# Autodesk Inventor assembly: Arm 2.0 Assembly
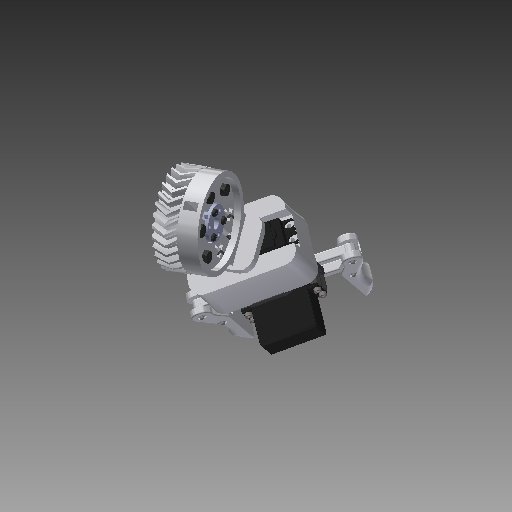
[picture p0: Inventor's stored thumbnail of the model, 512x512]
Saved by Autodesk Inventor 2017 (Build 210142000, 142)
## iProperties
Created: 2017-09-28
Part Number: Arm 2.0 Assembly
Document SubType Name: Assembly
Designer: Zach
Author: Zach
## Documents named in this file (13)
- C:\Users\Dell\Documents\GitHub\tr1\src\Body\Arm Assembly\End Effector Assembly\End Effector Assembly.iam
- C:\Users\Dell\Documents\GitHub\tr1\src\Body\Arm Assembly\End Effector Assembly\Gripper Assembly\Gripper B Assembly.iam
- C:\Users\Dell\Documents\GitHub\tr1\lib\8mm Hub.ipt
- C:\Users\Dell\Documents\GitHub\tr1\lib\Content Center Files\R2017\en-US\ISO 7045  H\ISO 7045 - M3 x 8 - 4.8 - H - ISO.ipt
- C:\Users\Dell\Documents\GitHub\tr1\src\Body\Arm Assembly\End Effector Assembly\AA046.ipt
- C:\Users\Dell\Documents\GitHub\tr1\lib\MG995.ipt
- C:\Users\Dell\Documents\GitHub\tr1\lib\Servo Mounting Hub.ipt
- C:\Users\Dell\Documents\GitHub\tr1\src\Body\Arm Assembly\End Effector Assembly\AA047.ipt
- C:\Users\Dell\Documents\GitHub\tr1\src\Body\Arm Assembly\End Effector Assembly\AA048.ipt
- C:\Users\Dell\Documents\GitHub\tr1\lib\Content Center Files\R2017\en-US\ISO 4018\ISO 4018 - M5 x 10.ipt
- C:\Users\Dell\Documents\GitHub\tr1\lib\Content Center Files\R2017\en-US\ISO 4018\ISO 4018 - M5 x 25.ipt
- C:\Users\Dell\Documents\GitHub\tr1\lib\Content Center Files\R2017\en-US\ISO 7045  H\ISO 7045 - M3 x 12 - 4.8 - H - ISO.ipt
- C:\Users\Dell\Documents\GitHub\tr1\src\Body\Arm Assembly\End Effector Assembly\AASG09b.ipt
## Components (22 placed, 12 different names)
1. AA046:1 — Mate:727, Mate:728, Mate:735, Mate:736, Mate:737, Mate:752, Mate:756, Mate:760, Mate:1298, Mate:1299, Mate:1300, Mate:1301, Mate:1302, Mate:1303, Mate:1304, Mate:1305
2. AA047:1 — Mate:735, Mate:736, Mate:737, Mate:738, Mate:739, Mate:740, Mate:753, Mate:754, Mate:755, Mate:800, Mate:801
3. AA048:1 — Mate:744, Mate:745, Mate:746, Mate:747, Mate:748, Mate:749
4. Gripper B Assembly:1 [sub-assembly] — Mate:747, Mate:748, Mate:749
5. 8mm Hub:9 — Mate:727, Mate:728, Mate:756, Mate:764, Mate:765, Mate:766, Mate:767, Mate:768, Mate:769
6. Servo Mounting Hub:1 — Mate:733, Mate:734, Mate:738, Mate:739, Mate:740, Mate:792, Mate:793, Mate:794, Mate:795, Mate:796, Mate:797, Mate:798, Mate:799
7. MG995:1 — Mate:733, Mate:734, Mate:744, Mate:745, Mate:746
8. ISO 7045 H M3 x 8 - 4.8 - H:7 — Mate:795, Mate:799
9. ISO 7045 H M3 x 8 - 4.8 - H:8 — Mate:794, Mate:798
10. ISO 7045 H M3 x 8 - 4.8 - H:9 — Mate:792, Mate:796
11. ISO 7045 H M3 x 8 - 4.8 - H:10 — Mate:793, Mate:797
12. ISO 7045 H M3 x 8 - 4.8 - H:11 — Mate:800, Mate:801
13. ISO 7045 H M3 x 12 - 4.8 - H:1 — Mate:765, Mate:767
14. ISO 7045 H M3 x 12 - 4.8 - H:3 — Mate:764, Mate:769
15. ISO 7045 H M3 x 12 - 4.8 - H:2 — Mate:766, Mate:768
16. ISO 4018 M5 x 10:1 — Mate:754, Mate:755
17. ISO 4018 M5 x 10:2 — Mate:752, Mate:753
18. ISO 4018 M5 x 25:1 — Mate:1299, Mate:1300
19. ISO 4018 M5 x 25:2 — Mate:1298, Mate:1301, Mate:1306
20. ISO 4018 M5 x 25:3 — Mate:760, Mate:1302
21. ISO 4018 M5 x 25:7 — Mate:1303, Mate:1304, Mate:1307
22. Spur Gear1:1 — Mate:1305, Mate:1306, Mate:1307
## Relationships (48: Mate 48)
- Mate:727: AA046:1 ↔ 8mm Hub:9
- Mate:728: AA046:1 ↔ 8mm Hub:9
- Mate:733: Servo Mounting Hub:1 ↔ MG995:1
- Mate:734: Servo Mounting Hub:1 ↔ MG995:1
- Mate:735: AA046:1 ↔ AA047:1
- Mate:736: AA046:1 ↔ AA047:1
- Mate:737: AA046:1 ↔ AA047:1
- Mate:738: AA047:1 ↔ Servo Mounting Hub:1
- Mate:739: AA047:1 ↔ Servo Mounting Hub:1
- Mate:740: AA047:1 ↔ Servo Mounting Hub:1
- Mate:744: AA048:1 ↔ MG995:1
- Mate:745 (0.5 mm): AA048:1 ↔ MG995:1
- Mate:746 (0.5 mm): AA048:1 ↔ MG995:1
- Mate:747: AA048:1 ↔ Gripper B Assembly:1
- Mate:748: AA048:1 ↔ Gripper B Assembly:1
- Mate:749: AA048:1 ↔ Gripper B Assembly:1
- Mate:752: AA046:1 ↔ ISO 4018 M5 x 10:2
- Mate:753: AA047:1 ↔ ISO 4018 M5 x 10:2
- Mate:754: AA047:1 ↔ ISO 4018 M5 x 10:1
- Mate:755: AA047:1 ↔ ISO 4018 M5 x 10:1
- Mate:756: AA046:1 ↔ 8mm Hub:9
- Mate:760: AA046:1 ↔ ISO 4018 M5 x 25:3
- Mate:764: 8mm Hub:9 ↔ ISO 7045 H M3 x 12 - 4.8 - H:3
- Mate:765: 8mm Hub:9 ↔ ISO 7045 H M3 x 12 - 4.8 - H:1
- Mate:766: 8mm Hub:9 ↔ ISO 7045 H M3 x 12 - 4.8 - H:2
- Mate:767: 8mm Hub:9 ↔ ISO 7045 H M3 x 12 - 4.8 - H:1
- Mate:768: 8mm Hub:9 ↔ ISO 7045 H M3 x 12 - 4.8 - H:2
- Mate:769: 8mm Hub:9 ↔ ISO 7045 H M3 x 12 - 4.8 - H:3
- Mate:792: Servo Mounting Hub:1 ↔ ISO 7045 H M3 x 8 - 4.8 - H:9
- Mate:793: Servo Mounting Hub:1 ↔ ISO 7045 H M3 x 8 - 4.8 - H:10
- Mate:794: Servo Mounting Hub:1 ↔ ISO 7045 H M3 x 8 - 4.8 - H:8
- Mate:795: Servo Mounting Hub:1 ↔ ISO 7045 H M3 x 8 - 4.8 - H:7
- Mate:796: Servo Mounting Hub:1 ↔ ISO 7045 H M3 x 8 - 4.8 - H:9
- Mate:797: Servo Mounting Hub:1 ↔ ISO 7045 H M3 x 8 - 4.8 - H:10
- Mate:798: Servo Mounting Hub:1 ↔ ISO 7045 H M3 x 8 - 4.8 - H:8
- Mate:799: Servo Mounting Hub:1 ↔ ISO 7045 H M3 x 8 - 4.8 - H:7
- Mate:800: AA047:1 ↔ ISO 7045 H M3 x 8 - 4.8 - H:11
- Mate:801: AA047:1 ↔ ISO 7045 H M3 x 8 - 4.8 - H:11
- Mate:1298: AA046:1 ↔ ISO 4018 M5 x 25:2
- Mate:1299: AA046:1 ↔ ISO 4018 M5 x 25:1
- Mate:1300: AA046:1 ↔ ISO 4018 M5 x 25:1
- Mate:1301: AA046:1 ↔ ISO 4018 M5 x 25:2
- Mate:1302: AA046:1 ↔ ISO 4018 M5 x 25:3
- Mate:1303: AA046:1 ↔ ISO 4018 M5 x 25:7
- Mate:1304: AA046:1 ↔ ISO 4018 M5 x 25:7
- Mate:1305: AA046:1 ↔ Spur Gear1:1
- Mate:1306: ISO 4018 M5 x 25:2 ↔ Spur Gear1:1
- Mate:1307: ISO 4018 M5 x 25:7 ↔ Spur Gear1:1
